# Autodesk Inventor assembly: DCJ11
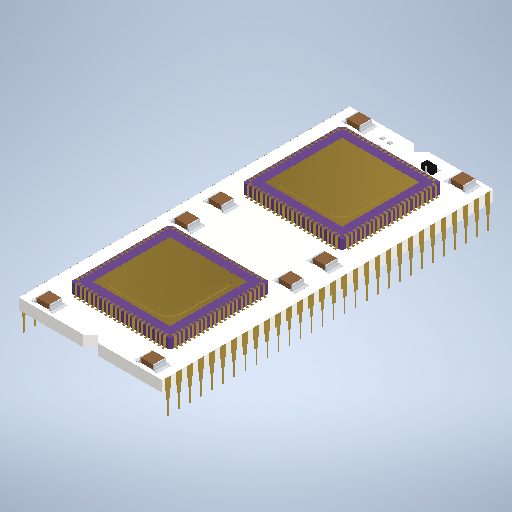
[picture p0: Inventor's stored thumbnail of the model, 512x512]
Saved by Autodesk Inventor 2025 (Build 290162000, 162)
## iProperties
Created: 2025-09-08
Part Number: DCJ11
Document SubType Name: Assembly
Designer: jirne
Author: jirne
## Documents named in this file (11)
- C:\Users\jirne\JVR11\hardware\library\3D\DCJ11\DCJ11.iam
- C:\Users\jirne\JVR11\hardware\library\3D\DCJ11\body.ipt
- C:\Users\jirne\JVR11\hardware\library\3D\DCJ11\pin.ipt
- C:\Users\jirne\JVR11\hardware\library\3D\DCJ11\chip\chip.iam
- C:\Users\jirne\JVR11\hardware\library\3D\DCJ11\capacitor\capacitor.iam
- C:\Users\jirne\JVR11\hardware\library\3D\DCJ11\capacitor\capacitor_MIR.iam
- C:\Users\jirne\JVR11\hardware\library\3D\DCJ11\bottom_plates.ipt
- C:\Users\jirne\JVR11\hardware\library\3D\DCJ11\bottom_plates_MIR.ipt
- C:\Users\jirne\JVR11\hardware\library\3D\DCJ11\transistor\connection_not_populated.ipt
- C:\Users\jirne\JVR11\hardware\library\3D\DCJ11\transistor\transistor.iam
- C:\Users\jirne\JVR11\hardware\library\3D\DCJ11\mark.ipt
## Components (83 placed, 10 different names)
1. chip:1 [sub-assembly] — Mate:3
2. chip:2 [sub-assembly]
3. body:1 — Mate:1, Mate:2, Mate:3, Mate:4, Mate:5, Mate:6, Mate:7, Mate:8, Mate:9, Mate:10, Mate:11
4. connection_not_populated:1 — Mate:4, Mate:5
5. transistor:1 [sub-assembly] — Mate:6, Mate:7
6. mark:1 — Mate:10, Mate:11
7. mark:2 — Mate:8, Mate:9
8. pin:1
9. pin:2
10. pin:3
11. pin:4
12. pin:5
13. pin:6
14. pin:7
15. pin:8
16. pin:9
17. pin:10
18. pin:11
19. pin:12
20. pin:13
21. pin:14
22. pin:15
23. pin:16
24. pin:17
25. pin:18
26. pin:19
27. pin:20
28. pin:21
29. pin:22
30. pin:23
31. pin:24
32. pin:25
33. pin:26
34. pin:27
35. pin:28
36. pin:29
37. pin:30
38. pin:31
39. pin:32
40. pin:33
41. pin:34
42. pin:35
43. pin:36
44. pin:37
45. pin:38
46. pin:39
47. pin:40
48. pin:41
49. pin:42
50. pin:43
51. pin:44
52. pin:45
53. pin:46
54. pin:47
55. pin:48
56. pin:49
57. pin:50
58. pin:51
59. pin:52
60. pin:53
61. pin:54
62. pin:55
63. pin:56
64. pin:57
65. pin:58
66. pin:59
67. pin:60
68. capacitor:1 [sub-assembly] — Mate:1, Mate:2
69. capacitor:2 [sub-assembly]
70. capacitor:3 [sub-assembly]
71. capacitor:4 [sub-assembly]
72. capacitor_MIR:1 [sub-assembly]
73. capacitor_MIR:2 [sub-assembly]
74. capacitor_MIR:3 [sub-assembly]
75. capacitor_MIR:4 [sub-assembly]
76. bottom_plates:1
77. bottom_plates:2
78. bottom_plates:3
79. bottom_plates:4
80. bottom_plates_MIR:1
81. bottom_plates_MIR:2
82. bottom_plates_MIR:3
83. bottom_plates_MIR:4
## Component patterns: (30 elements, first: pin:1), (30 elements, first: pin:31), (4 elements, first: capacitor:1), (4 elements, first: capacitor_MIR:1), (4 elements, first: bottom_plates:1), (4 elements, first: bottom_plates_MIR:1)
## Relationships (11: Mate 11)
- Mate:1: body:1 ↔ capacitor:1
- Mate:2: body:1 ↔ capacitor:1
- Mate:3: chip:1 ↔ body:1
- Mate:4: body:1 ↔ connection_not_populated:1
- Mate:5: body:1 ↔ connection_not_populated:1
- Mate:6: body:1 ↔ transistor:1
- Mate:7: body:1 ↔ transistor:1
- Mate:8: body:1 ↔ mark:2
- Mate:9: body:1 ↔ mark:2
- Mate:10: body:1 ↔ mark:1
- Mate:11: body:1 ↔ mark:1
